# Autodesk Inventor assembly: Motor_pulley_assembly
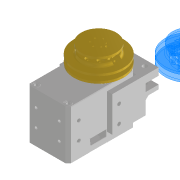
[picture p0: Inventor's stored thumbnail of the model, 180x180]
Saved by Autodesk Inventor 2022 (Build 260153000, 153)
## iProperties
Created: 2022-07-09
Part Number: Motor_pulley_assembly
Document SubType Name: Assembly
Designer: dell
Author: dell
## Documents named in this file (4)
- D:\xxxx\Uni\Part IV\MECHENG_700\Part_IV_project_CAD\Bird_skeleton_prototypes\Wing_drone_V1\Bird_wing_V2\Motor_pulley_assembly.iam
- D:\xxxx\Uni\Part IV\MECHENG_700\Part_IV_project_CAD\Bird_skeleton_prototypes\Wing_drone_V1\XM430.iam
- D:\xxxx\Uni\Part IV\MECHENG_700\Part_IV_project_CAD\Bird_skeleton_prototypes\Wing_drone_V1\Bird_wing_V2\Motor_pulley.ipt
- D:\xxxx\Uni\Part IV\MECHENG_700\Part_IV_project_CAD\Bird_skeleton_prototypes\Wing_drone_V1\Bird_wing_V2\Wing_shoulder\Bar_motor_mount.ipt
## Components (3 placed, 3 different names)
1. XM430:1 [sub-assembly] — Mate:5, Mate:6, Mate:7, Mate:8, Mate:9, Mate:10
2. Motor_pulley:1 — Mate:9, Mate:10
3. Bar_motor_mount:1 — Mate:5, Mate:6, Mate:7, Mate:8
## Relationships (6: Mate 6)
- Mate:5: XM430:1 ↔ Bar_motor_mount:1
- Mate:6: XM430:1 ↔ Bar_motor_mount:1
- Mate:7: XM430:1 ↔ Bar_motor_mount:1
- Mate:8 (0.25 mm): XM430:1 ↔ Bar_motor_mount:1
- Mate:9: XM430:1 ↔ Motor_pulley:1
- Mate:10: XM430:1 ↔ Motor_pulley:1
